# Autodesk Inventor assembly: Stewart-Sym-Base
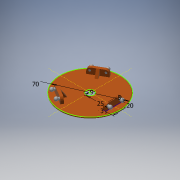
[picture p0: Inventor's stored thumbnail of the model, 180x180]
Saved by Autodesk Inventor 2018.2 (Build 222227000, 227)
## iProperties
Created: 2018-03-01
Part Number: Stewart-Sym-Base
Material: Generisch
Document SubType Name: Assembly
Designer: JochenAlt
Author: JochenAlt
## Documents named in this file (3)
- D:\Projects\Donna\CAD\KST DS215MG\Stewart-Sym-Base.iam
- D:\Projects\Donna\CAD\KST DS215MG\Stewart-Sym-Base.ipt
- D:\Projects\Donna\CAD\KST DS215MG\Ball-Joint-male.ipt
## Components (7 placed, 2 different names)
1. Stewart-Plate-Head:1 — Passend:1, Passend:2, Passend:3, Passend:4, Passend:5, Passend:6, Passend:7, Passend:8, Passend:9, Passend:10, Passend:11, Passend:12, Passend:13, Passend:14, Passend:15
2. ball joint:1 — Passend:4, Passend:12
3. ball joint:2 — Passend:9, Passend:15
4. ball joint:3 — Passend:6, Passend:14
5. ball joint:4 — Passend:5, Passend:13
6. ball joint:5 — Passend:7, Passend:11
7. ball joint:6 — Passend:8, Passend:10
## Relationships (15: Mate 15)
- Passend:1 [Mate]: Stewart-Plate-Head:1
- Passend:2 [Mate]: Stewart-Plate-Head:1
- Passend:3 [Mate]: Stewart-Plate-Head:1
- Passend:4 [Mate]: Stewart-Plate-Head:1 ↔ ball joint:1
- Passend:5 [Mate]: Stewart-Plate-Head:1 ↔ ball joint:4
- Passend:6 [Mate]: Stewart-Plate-Head:1 ↔ ball joint:3
- Passend:7 [Mate]: Stewart-Plate-Head:1 ↔ ball joint:5
- Passend:8 [Mate]: Stewart-Plate-Head:1 ↔ ball joint:6
- Passend:9 [Mate]: Stewart-Plate-Head:1 ↔ ball joint:2
- Passend:10 [Mate]: Stewart-Plate-Head:1 ↔ ball joint:6
- Passend:11 [Mate]: Stewart-Plate-Head:1 ↔ ball joint:5
- Passend:12 [Mate]: Stewart-Plate-Head:1 ↔ ball joint:1
- Passend:13 [Mate]: Stewart-Plate-Head:1 ↔ ball joint:4
- Passend:14 [Mate]: Stewart-Plate-Head:1 ↔ ball joint:3
- Passend:15 [Mate]: Stewart-Plate-Head:1 ↔ ball joint:2
